# Autodesk Inventor assembly: 000.001 - Куб типа Э (красный)
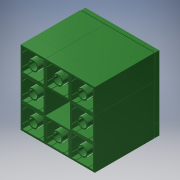
[picture p0: Inventor's stored thumbnail of the model, 180x180]
Saved by Autodesk Inventor 2019 (Build 230136000, 136)
## iProperties
Created: 2020-02-29
Part Number: 000.001 - Куб типа Э (красный)
Material: Типовые
Document SubType Name: Assembly
Designer: Петров Иван
Author: Петров Иван
## Documents named in this file (4)
- E:\IVAN\Ivan_desktop\GitHub\Manipulation_IRS\hardware\000.001 - Куб типа Э (зеленый).iam
- E:\IVAN\Ivan_desktop\GitHub\Manipulation_IRS\hardware\components\modular-lego-brick-standard-1.snapshot.7\Brick standard 4x2.ipt
- E:\IVAN\Ivan_desktop\GitHub\Manipulation_IRS\hardware\components\modular-lego-brick-standard-1.snapshot.7\1x4 flat RED.ipt
- E:\IVAN\Ivan_desktop\GitHub\Manipulation_IRS\hardware\components\modular-lego-brick-standard-1.snapshot.7\Brick standard 2x2.ipt
## Components (25 placed, 3 different names)
1. Brick standard 2x2:1 — Совмещение:6, Совмещение:7, Заподлицо:11
2. Brick standard 4x2:2 — Совмещение:1, Заподлицо:1, Заподлицо:2, Заподлицо:6
3. Brick standard 4x2:4 — Заподлицо:5, Совмещение:3, Заподлицо:6
4. Brick standard 4x2:1 — Совмещение:1, Заподлицо:1, Заподлицо:2, Совмещение:2, Заподлицо:3, Заподлицо:4
5. Brick standard 4x2:3 — Совмещение:2, Заподлицо:3, Заподлицо:4, Заподлицо:5, Совмещение:3
6. Brick standard 4x2:5
7. Brick standard 4x2:6
8. Brick standard 4x2:7
9. Brick standard 4x2:8
10. Brick standard 4x2:9
11. Brick standard 4x2:10
12. Brick standard 4x2:11
13. Brick standard 4x2:12
14. Brick standard 4x2:13 — Заподлицо:8, Заподлицо:9
15. Brick standard 4x2:14 — Заподлицо:7, Совмещение:4
16. Brick standard 4x2:15 — Совмещение:7, Заподлицо:11
17. Brick standard 4x2:16 — Совмещение:6
18. 1x4 flat RED:2 — Заподлицо:7, Совмещение:4, Заподлицо:8, Заподлицо:10, Совмещение:5
19. 1x4 flat RED:1 — Заподлицо:9, Заподлицо:10, Совмещение:5
20. 1x4 flat RED:3
21. 1x4 flat RED:4
22. 1x4 flat RED:5
23. 1x4 flat RED:6
24. 1x4 flat RED:7
25. 1x4 flat RED:8
## Component patterns: (4 elements, first: Brick standard 4x2:2 + Brick standard 4x2:4 + Brick standard 4x2:1 + Brick standard 4x2:3), (4 elements, first: 1x4 flat RED:2 + 1x4 flat RED:1)
## Relationships (18: Flush 11, Mate 7)
- Совмещение:1 [Mate]: Brick standard 4x2:2 ↔ Brick standard 4x2:1
- Заподлицо:1 [Flush]: Brick standard 4x2:2 ↔ Brick standard 4x2:1
- Заподлицо:2 [Flush]: Brick standard 4x2:2 ↔ Brick standard 4x2:1
- Совмещение:2 [Mate]: Brick standard 4x2:1 ↔ Brick standard 4x2:3
- Заподлицо:3 [Flush]: Brick standard 4x2:1 ↔ Brick standard 4x2:3
- Заподлицо:4 [Flush]: Brick standard 4x2:1 ↔ Brick standard 4x2:3
- Заподлицо:5 [Flush]: Brick standard 4x2:4 ↔ Brick standard 4x2:3
- Совмещение:3 [Mate]: Brick standard 4x2:4 ↔ Brick standard 4x2:3
- Заподлицо:6 [Flush]: Brick standard 4x2:2 ↔ Brick standard 4x2:4
- Заподлицо:7 [Flush]: Brick standard 4x2:14 ↔ 1x4 flat RED:2
- Совмещение:4 [Mate]: Brick standard 4x2:14 ↔ 1x4 flat RED:2
- Заподлицо:8 [Flush]: Brick standard 4x2:13 ↔ 1x4 flat RED:2
- Заподлицо:9 [Flush]: Brick standard 4x2:13 ↔ 1x4 flat RED:1
- Заподлицо:10 [Flush]: 1x4 flat RED:2 ↔ 1x4 flat RED:1
- Совмещение:5 [Mate]: 1x4 flat RED:2 ↔ 1x4 flat RED:1
- Совмещение:6 [Mate]: Brick standard 2x2:1 ↔ Brick standard 4x2:16
- Совмещение:7 [Mate]: Brick standard 2x2:1 ↔ Brick standard 4x2:15
- Заподлицо:11 [Flush]: Brick standard 2x2:1 ↔ Brick standard 4x2:15
